# Autodesk Inventor assembly: FingerGeneric
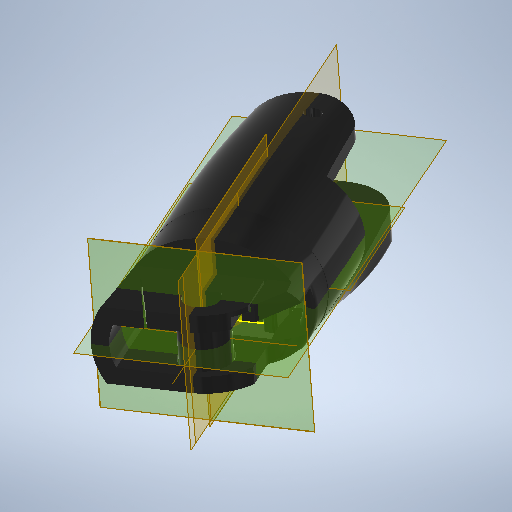
[picture p0: Inventor's stored thumbnail of the model, 512x512]
Saved by Autodesk Inventor 2025.1 (Build 291241000, 241)
## iProperties
Created: 2024-09-11
Part Number: FingerGeneric
Document SubType Name: Assembly
Designer: Alexander
Mass: 5.58048 g
Surface Area: 47.3633 cm^2
Volume: 4.35975 cm^3
Density: 1.28 g/cm^3
Author: Alexander
## Documents named in this file (4)
- D:\Repositorios_Politecnica\Handi-EPN\CAD\Sim Models\GenericProximalPhalanx.iam
- D:\Repositorios_Politecnica\Handi-EPN\CAD\Right Finger\PP - P MainD2 R.ipt
- D:\Repositorios_Politecnica\Handi-EPN\CAD\Right Finger\PP - P PivotD2 R.ipt
- D:\Repositorios_Politecnica\Handi-EPN\CAD\Right Finger\PP - D R.ipt
## Components (3 placed, 3 different names)
1. PP - P MainD2 R:1 — Mate:2, Flush:3, Flush:4, Cylindrical:1, Flush:5, Symmetry:1, Flush:7, Flush:8
2. PP - P PivotD2 R:1 — Cylindrical:1, Flush:5, Symmetry:1
3. PP - D R:1 — Mate:2, Flush:3, Flush:4
## Relationships (9: Flush 6, Mate 1, CylindricalJoint 1, Symmetry 1)
- Mate:2: PP - P MainD2 R:1 ↔ PP - D R:1
- Flush:3: PP - P MainD2 R:1 ↔ PP - D R:1
- Flush:4 (2.3 mm): PP - P MainD2 R:1 ↔ PP - D R:1
- Cylindrical:1: PP - P MainD2 R:1 ↔ PP - P PivotD2 R:1
- Flush:5: PP - P MainD2 R:1 ↔ PP - P PivotD2 R:1
- Symmetry:1: PP - P MainD2 R:1 ↔ PP - P PivotD2 R:1
- Flush:6
- Flush:7: PP - P MainD2 R:1
- Flush:8: PP - P MainD2 R:1
